# Autodesk Inventor assembly: Assembly1
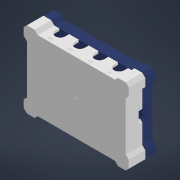
[picture p0: Inventor's stored thumbnail of the model, 180x180]
Saved by Autodesk Inventor 2021.4 (Build 254397000, 397)
## iProperties
Created: 2022-03-02
Part Number: Assembly1
Document SubType Name: Assembly
Designer: Alex
Author: Alex
## Documents named in this file (3)
- C:\Users\Alex\3D Objects\Inventor\Omniplex\Assembly1.iam
- C:\Users\Alex\3D Objects\Inventor\Omniplex\Case.ipt
- C:\Users\Alex\3D Objects\Inventor\Omniplex\Lid.ipt
## Components (2 placed, 2 different names)
1. Case:1 — Flush:1
2. Lid:1 — Flush:1
## Relationships (1: Flush 1)
- Flush:1: Case:1 ↔ Lid:1
